# Autodesk Inventor assembly: test_assy
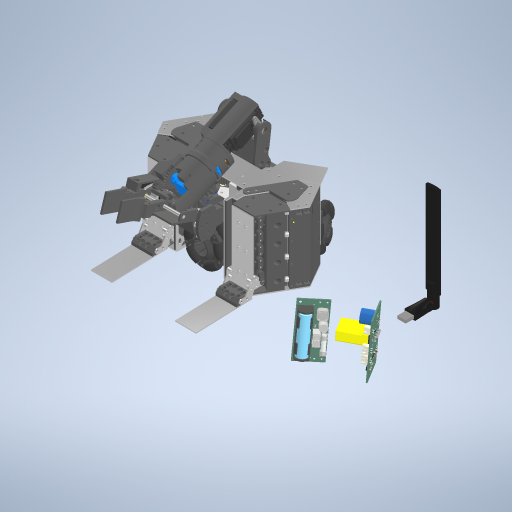
[picture p0: Inventor's stored thumbnail of the model, 512x512]
Saved by Autodesk Inventor 2024.1 (Build 281209000, 209)
## iProperties
Created: 2025-01-17
Part Number: test_assy
Document SubType Name: Assembly
Designer: hibik
Author: hibik
## Documents named in this file (8)
- C:\Users\hibik\Documents\Robomech\RESCUE\ORCA\hard\test_assy.iam
- C:\Users\hibik\Documents\Robomech\RESCUE\ORCA\hard\camera\cam_set.iam
- C:\Users\hibik\Documents\Robomech\RESCUE\ORCA\hard\std_parts\Buffalo_Wl-U2-433DHP.ipt
- C:\Users\hibik\Documents\Robomech\RESCUE\ORCA\hard\cover.ipt
- C:\Users\hibik\Documents\Robomech\RESCUE\ORCA\hard\arm\Assy_arm.iam
- C:\Users\hibik\Documents\Robomech\RESCUE\ORCA\hard\Assy_fork_connection.iam
- C:\Users\hibik\Documents\Robomech\RESCUE\ORCA\hard\board\core_power.iam
- C:\Users\hibik\Documents\Robomech\RESCUE\ORCA\hard\board\core_usp.iam
## Components (7 placed, 7 different names)
1. cam_set:1 [sub-assembly] — フラッシュ:4, 角度:8
2. Buffalo_Wl-U2-433DHP:1
3. cover:1 — フラッシュ:8, フラッシュ:9, フラッシュ:10
4. Assy_fork_connection:1 [sub-assembly] — フラッシュ:11, メイト:6, メイト:7
5. Assy_arm:1 [sub-assembly] — フラッシュ:11, メイト:6, メイト:7
6. core_power:1 [sub-assembly]
7. core_usp:1 [sub-assembly]
## Relationships (13: Flush 6, Mate 4, Angle 3)
- メイト:4 [Mate]
- 角度:6 [Angle] (60 deg)
- メイト:5 [Mate]
- 角度:7 [Angle] (-60 deg)
- フラッシュ:4 [Flush] (-26.9 mm): cam_set:1
- フラッシュ:5 [Flush] (100 mm)
- 角度:8 [Angle] (0 deg): cam_set:1
- フラッシュ:8 [Flush]: cover:1
- フラッシュ:9 [Flush]: cover:1
- フラッシュ:10 [Flush]: cover:1
- フラッシュ:11 [Flush]: Assy_fork_connection:1 ↔ Assy_arm:1
- メイト:6 [Mate] (15 mm): Assy_fork_connection:1 ↔ Assy_arm:1
- メイト:7 [Mate] (1 mm): Assy_fork_connection:1 ↔ Assy_arm:1
